# Autodesk Inventor assembly: Medium Conveyor-Belt Link
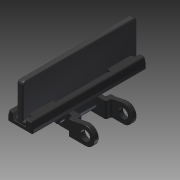
[picture p0: Inventor's stored thumbnail of the model, 180x180]
Saved by Autodesk Inventor 2015 SP1 (Build 190201100, 201)
## iProperties
Category: Motion
Company: Super Sonic Sparks, Team 24
Vendor: VEX Robotics, Inc.
Document SubType Name: Assembly
Designer: Jordan Kiesel
Catalog Web Link: vexrobotics.com/276-2214.html
Description: For use in constructing conveyor belt type mechanisms.
Mass: 2.59824 g
Surface Area: 29.3637 cm^2
Volume: 2.17651 cm^3
Density: 1.19377 g/cm^3
Author: Jordan Kiesel
Title: Medium Conveyor-Belt Link
Comments: For use in constructing conveyor belt type mechanisms. ▷ Compatible with Tank Tread Kit, High Strength Chain & Sprockets.
## Documents named in this file (3)
- C:\Users\Jordan\Documents\Robotics\VEX\CAD\2015 BNS CAD Library (beta)\Motion\Chain & Tank Tread\Short Conveyor-Belt Link.iam
- C:\Users\Jordan\Documents\Robotics\VEX\CAD\2015 BNS CAD Library (beta)\Motion\Chain & Tank Tread\Reference Parts\Conveyor-Belt Links\Conveyor-Belt Base Link.ipt
- C:\Users\Jordan\Documents\Robotics\VEX\CAD\2015 BNS CAD Library (beta)\Motion\Chain & Tank Tread\Reference Parts\Conveyor-Belt Links\Short Conveyor-Belt Insert.ipt
## Components (2 placed, 2 different names)
1. Conveyor-Belt Base Link:1 — Mate:1, Mate:2, Flush:1
2. Short Conveyor-Belt Insert:1 — Mate:1, Mate:2, Flush:1
## Relationships (3: Mate 2, Flush 1)
- Mate:1: Conveyor-Belt Base Link:1 ↔ Short Conveyor-Belt Insert:1
- Mate:2: Conveyor-Belt Base Link:1 ↔ Short Conveyor-Belt Insert:1
- Flush:1: Conveyor-Belt Base Link:1 ↔ Short Conveyor-Belt Insert:1
